# Autodesk Inventor assembly: TZS 0970 top funnel
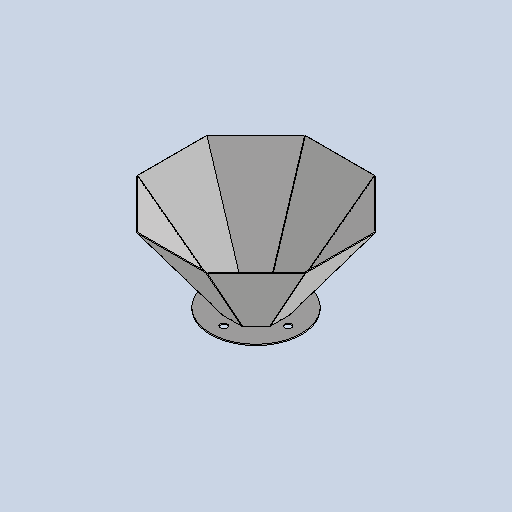
[picture p0: Inventor's stored thumbnail of the model, 512x512]
Saved by Autodesk Inventor 2025.3 (Build 293356030, 356C)
## iProperties
Created: 2025-07-11
Part Number: TZS 0970 top funnel
Document SubType Name: Assembly
Designer: user
Author: user
## Documents named in this file (3)
- C:\Users\admin\Yandex.Disk\home pc\Inventor\ANP--Antipayuta\FDS 1400\воронка\TZS 0970 top funnel.iam
- C:\Users\admin\Yandex.Disk\home pc\Inventor\ANP--Antipayuta\FDS 1400\воронка\TZS 0971 top funnel wall.ipt
- C:\Users\admin\Yandex.Disk\home pc\Inventor\ANP--Antipayuta\FDS 1400\воронка\TZS 0972 funnel FLANGE 50-90.ipt
## Components (3 placed, 2 different names)
1. TZS 0972 funnel FLANGE 50-90.ipt:1 — Mate:1, Mate:2, Mate:3, Mate:4, Mate:6, Mate:7
2. TZS 0971 top funnel wall.ipt:1 — Mate:1, Mate:2, Mate:5, Mate:7
3. TZS 0971 top funnel wall.ipt:2 — Mate:3, Mate:4, Mate:5, Mate:6
## Relationships (7: Mate 7)
- Mate:1: TZS 0972 funnel FLANGE 50-90.ipt:1 ↔ TZS 0971 top funnel wall.ipt:1
- Mate:2: TZS 0972 funnel FLANGE 50-90.ipt:1 ↔ TZS 0971 top funnel wall.ipt:1
- Mate:3: TZS 0972 funnel FLANGE 50-90.ipt:1 ↔ TZS 0971 top funnel wall.ipt:2
- Mate:4: TZS 0972 funnel FLANGE 50-90.ipt:1 ↔ TZS 0971 top funnel wall.ipt:2
- Mate:5: TZS 0971 top funnel wall.ipt:1 ↔ TZS 0971 top funnel wall.ipt:2
- Mate:6 (-2.87 mm): TZS 0972 funnel FLANGE 50-90.ipt:1 ↔ TZS 0971 top funnel wall.ipt:2
- Mate:7 (-2.87 mm): TZS 0972 funnel FLANGE 50-90.ipt:1 ↔ TZS 0971 top funnel wall.ipt:1
